# Autodesk Inventor assembly: main_assembly
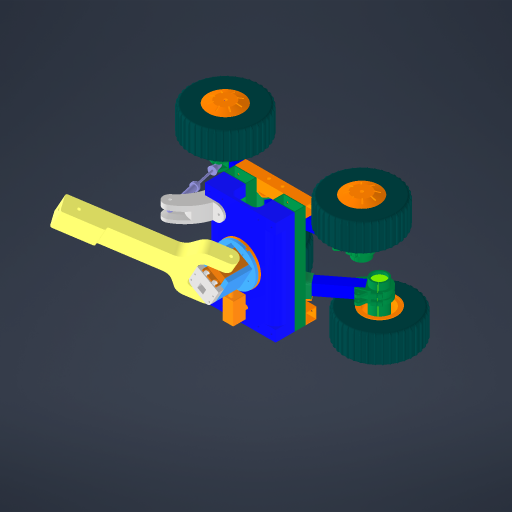
[picture p0: Inventor's stored thumbnail of the model, 512x512]
Saved by Autodesk Inventor 2024 (Build 280153000, 153)
## iProperties
Created: 2023-09-26
Part Number: main_assembly
Document SubType Name: Assembly
Designer: user
Author: user
## Documents named in this file (10)
- D:\Docs\Robot\3d_v2\main_assembly.iam
- D:\Docs\Robot\3d_v2\base\base_assambly.iam
- D:\Docs\Robot\3d_v2\machine_body\arm_assembly_r.iam
- D:\Docs\Robot\3d_v2\machine_body\arm_assembly_l.iam
- D:\Docs\Robot\3d_v2\electronics\Battery_18650_asembly.iam
- D:\Docs\Robot\3d_v2\electronics\Arduino MEGA 2560 R3.ipt
- D:\Docs\Robot\3d_v2\electronics\BTS7960\BTS7960.iam
- D:\Docs\Robot\3d_v2\machine_body\manipulator.iam
- D:\Docs\Robot\3d_v2\machine_body\shok_absorber_holder\shock_absorber_holder.ipt
- D:\Docs\Robot\3d_v2\default_components\shock_absorber.ipt
## Components (12 placed, 9 different names)
1. base_assambly:1 [sub-assembly] — Совмещение:1, Совмещение:2, Совмещение:3, Заподлицо:1, Заподлицо:2, Совмещение:4, Вставка:1, Вставка:3, Вставка:4, Вставка:5
2. Battery_18650_asembly:1 [sub-assembly]
3. Arduino MEGA 2560 R3:1
4. BTS7960:1 [sub-assembly]
5. BTS7960:2 [sub-assembly]
6. manipulator:1 [sub-assembly] — Заподлицо:1, Заподлицо:2, Совмещение:4, Заподлицо:3
7. arm_assembly_r:1 [sub-assembly] — Вставка:1
8. arm_assembly_r:2 [sub-assembly] — Вставка:5
9. arm_assembly_l:1 [sub-assembly] — Вставка:4
10. arm_assembly_l:2 [sub-assembly] — Вставка:3, Вставка:7
11. shock_absorber_holder:1 — Заподлицо:3, Вставка:8
12. shock_absorber:1 — Вставка:7, Вставка:8
## Relationships (13: Insert 6, Mate 4, Flush 3)
- Совмещение:1 [Mate]: base_assambly:1
- Совмещение:2 [Mate]: base_assambly:1
- Совмещение:3 [Mate]: base_assambly:1
- Заподлицо:1 [Flush]: base_assambly:1 ↔ manipulator:1
- Заподлицо:2 [Flush]: base_assambly:1 ↔ manipulator:1
- Совмещение:4 [Mate]: base_assambly:1 ↔ manipulator:1
- Вставка:1 [Insert]: base_assambly:1 ↔ arm_assembly_r:1
- Вставка:3 [Insert]: base_assambly:1 ↔ arm_assembly_l:2
- Вставка:4 [Insert]: base_assambly:1 ↔ arm_assembly_l:1
- Вставка:5 [Insert]: base_assambly:1 ↔ arm_assembly_r:2
- Заподлицо:3 [Flush]: manipulator:1 ↔ shock_absorber_holder:1
- Вставка:7 [Insert]: arm_assembly_l:2 ↔ shock_absorber:1
- Вставка:8 [Insert]: shock_absorber_holder:1 ↔ shock_absorber:1
